# Autodesk Inventor assembly: ASY PNS 179 top funnel 1200 50-90_1600
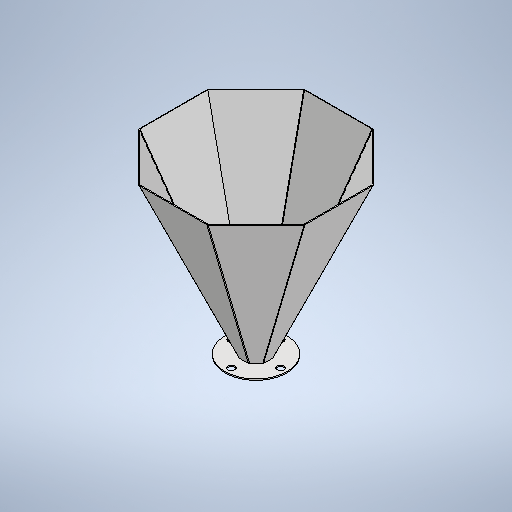
[picture p0: Inventor's stored thumbnail of the model, 512x512]
Saved by Autodesk Inventor 2025.1 (Build 291241020, 241B)
## iProperties
Created: 2025-07-11
Part Number: ASY PNS 179 top funnel 1200 50-90_1600
Document SubType Name: Assembly
Designer: user
Author: user
## Documents named in this file (3)
- C:\Users\user\YandexDisk-badmisterfox\home pc\Inventor\PNS2-Panaevsk\Filter D1200\ASY PNS 179 top funnel 1200 50-90_1600.iam
- C:\Users\user\YandexDisk-badmisterfox\home pc\Inventor\PNS2-Panaevsk\filter-distribution-system\PNS 1792  funnel FLANGE 1200 50-90_1600.ipt
- C:\Users\user\YandexDisk-badmisterfox\home pc\Inventor\PNS2-Panaevsk\Filter D1200\PNS 1791 top funnel 1200 50-90_1600.ipt
## Components (3 placed, 2 different names)
1. PNS 1792  funnel FLANGE 1200 50-90_1600:1 — Mate:7, Mate:2, Mate:1, Mate:6, Mate:4, Mate:3
2. PNS 1791 top funnel 1200 50-90_1600:1 — Mate:7, Mate:2, Mate:1, Mate:5
3. PNS 1791 top funnel 1200 50-90_1600:2 — Mate:6, Mate:5, Mate:4, Mate:3
## Relationships (7: Mate 7)
- Mate:7 (-2.5 mm): PNS 1792  funnel FLANGE 1200 50-90_1600:1 ↔ PNS 1791 top funnel 1200 50-90_1600:1
- Mate:2: PNS 1792  funnel FLANGE 1200 50-90_1600:1 ↔ PNS 1791 top funnel 1200 50-90_1600:1
- Mate:1: PNS 1792  funnel FLANGE 1200 50-90_1600:1 ↔ PNS 1791 top funnel 1200 50-90_1600:1
- Mate:6 (-2.5 mm): PNS 1792  funnel FLANGE 1200 50-90_1600:1 ↔ PNS 1791 top funnel 1200 50-90_1600:2
- Mate:5: PNS 1791 top funnel 1200 50-90_1600:1 ↔ PNS 1791 top funnel 1200 50-90_1600:2
- Mate:4: PNS 1792  funnel FLANGE 1200 50-90_1600:1 ↔ PNS 1791 top funnel 1200 50-90_1600:2
- Mate:3: PNS 1792  funnel FLANGE 1200 50-90_1600:1 ↔ PNS 1791 top funnel 1200 50-90_1600:2
